# Autodesk Inventor assembly: Idler Pulley Assm - Nylon Spacer - Bolt
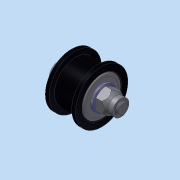
[picture p0: Inventor's stored thumbnail of the model, 180x180]
Saved by Autodesk Inventor 2013 (Build 170138000, 138)
## iProperties
Created: 2013-07-02
Part Number: Idler Pulley Assm - Nylon Spacer - Bolt
Document SubType Name: Assembly
Designer: Jon Hollander
Author: Jon Hollander
## Documents named in this file (7)
- D:\Dropbox\Research\CAD Library\v-slot\Part Assemblies\Idler Pulley - Spacer - Bolt\Workspaces\Workspace\Libary Import\Idler Bolt Assm\Idler Pulley Assm - Nylon Spacer - Bolt.iam
- D:\Dropbox\Research\CAD Library\v-slot\Part Assemblies\Idler Pulley - Spacer - Bolt\Libraries\Content Center Files\en-US\V-Slot Idler Pulley\V-Slot Idler Pulley.ipt
- D:\Dropbox\Research\CAD Library\v-slot\Part Assemblies\Idler Pulley - Spacer - Bolt\Libraries\Content Center Files\en-US\5mm Precision Washer\5mm Precision Washer.ipt
- D:\Dropbox\Research\CAD Library\v-slot\Part Assemblies\Idler Pulley - Spacer - Bolt\Libraries\Content Center Files\en-US\ANSI B18.16.3M(2)\ANSI B18.16.3M - Property Class 5 and 10 - Metric M5 x 0.8 Top Insert Type.ipt
- D:\Dropbox\Research\CAD Library\v-slot\Part Assemblies\Idler Pulley - Spacer - Bolt\Libraries\Content Center Files\en-US\One_Eighth_Nylon_Spacer_v2\Nylon Spacer 0.125.ipt
- D:\Dropbox\Research\CAD Library\v-slot\Part Assemblies\Idler Pulley - Spacer - Bolt\Libraries\Content Center Files\en-US\ANSI B18.3.4M(1)\ANSI B18.3.4M - M5 x 0.8 x 25(2).ipt
- D:\Dropbox\Research\CAD Library\v-slot\Bearing - 625 2RS\625 2RS Bearing.ipt
## Components (7 placed, 6 different names)
1. Broached Hexagon Socket Button Head Cap Screw - Metric M5 x 0.8 x 25:1 — Mate:9, Mate:11, Mate:15, Mate:19, Mate:21, Mate:23
2. V-Slot Idler Pulley V-Slot Idler Pulley:1 — Mate:23, Flush:1
3. 625 2RS Bearing:1 — Mate:19, Mate:20
4. 625 2RS Bearing:2 — Mate:21, Mate:22, Flush:1
5. 5mm Precision Washer 5mm Precision Washer:2 — Mate:9, Mate:18, Mate:20
6. Prevailing Torque Type Hex Nut - Steel Metric Property Class 5 and 10 - Metric M5 x 0.8 Top Insert Type:1 — Mate:11, Mate:18
7. One_Eighth_Nylon_Spacer_v2 Nylon Spacer 0.125:1 — Mate:15, Mate:22
## Relationships (12: Mate 11, Flush 1)
- [Mate]: Broached Hexagon Socket Button Head Cap Screw - Metric M5 x 0.8 x 25:1 ↔ 625 2RS Bearing:1
- [Mate]: Broached Hexagon Socket Button Head Cap Screw - Metric M5 x 0.8 x 25:1 ↔ 625 2RS Bearing:2
- Mate:9: Broached Hexagon Socket Button Head Cap Screw - Metric M5 x 0.8 x 25:1 ↔ 5mm Precision Washer 5mm Precision Washer:2
- Mate:15: Broached Hexagon Socket Button Head Cap Screw - Metric M5 x 0.8 x 25:1 ↔ One_Eighth_Nylon_Spacer_v2 Nylon Spacer 0.125:1
- Mate:18: 5mm Precision Washer 5mm Precision Washer:2 ↔ Prevailing Torque Type Hex Nut - Steel Metric Property Class 5 and 10 - Metric M5 x 0.8 Top Insert Type:1
- Mate:19: Broached Hexagon Socket Button Head Cap Screw - Metric M5 x 0.8 x 25:1 ↔ 625 2RS Bearing:1
- Mate:20: 625 2RS Bearing:1 ↔ 5mm Precision Washer 5mm Precision Washer:2
- Mate:21: Broached Hexagon Socket Button Head Cap Screw - Metric M5 x 0.8 x 25:1 ↔ 625 2RS Bearing:2
- Mate:22: 625 2RS Bearing:2 ↔ One_Eighth_Nylon_Spacer_v2 Nylon Spacer 0.125:1
- Mate:23: Broached Hexagon Socket Button Head Cap Screw - Metric M5 x 0.8 x 25:1 ↔ V-Slot Idler Pulley V-Slot Idler Pulley:1
- Flush:1 (0.2375 mm): V-Slot Idler Pulley V-Slot Idler Pulley:1 ↔ 625 2RS Bearing:2
- Mate:11: Broached Hexagon Socket Button Head Cap Screw - Metric M5 x 0.8 x 25:1 ↔ Prevailing Torque Type Hex Nut - Steel Metric Property Class 5 and 10 - Metric M5 x 0.8 Top Insert Type:1
